# Autodesk Inventor assembly: сборка основание
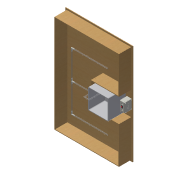
[picture p0: Inventor's stored thumbnail of the model, 180x180]
Saved by Autodesk Inventor 2021 (Build 250183000, 183)
## iProperties
Created: 2023-02-14
Part Number: сборка основание
Document SubType Name: Assembly
Designer: Tasya
Author: Tasya
## Documents named in this file (14)
- C:\Users\Tasya\Desktop\теплица\3D\Сборки iam\сборка основание.iam
- C:\Users\Tasya\Desktop\теплица\основание\основание.ipt
- C:\Users\Tasya\Desktop\теплица\основание\сосуд.ipt
- C:\Users\Tasya\Desktop\теплица\основание\стенка 1.ipt
- C:\Users\Tasya\Desktop\теплица\основание\стенка боковая.ipt
- C:\Users\Tasya\Desktop\теплица\основание\стенка 2.ipt
- C:\Users\Tasya\Desktop\теплица\основание\стенка 3.ipt
- C:\Users\Tasya\Desktop\теплица\основание\стенка 4.ipt
- C:\Users\Tasya\Desktop\теплица\емкость\шланг передний.ipt
- C:\Users\Tasya\Desktop\теплица\емкость\шланг боковой.ipt
- C:\Users\Tasya\Desktop\теплица\емкость\компановка емкость.iam
- C:\Users\Tasya\Desktop\теплица\емкость\змея.ipt
- C:\Users\Tasya\Desktop\теплица\емкость\соединитель 1.ipt
- C:\Users\Tasya\Desktop\теплица\емкость\соединитель 2.ipt
## Components (19 placed, 13 different names)
1. основание:1 — Угол:2, Угол:5, Заподлицо:1, Совмещение:50, Совмещение:51, Совмещение:54, Совмещение:55, Совмещение:56, Заподлицо:3, Совмещение:57, Совмещение:58, Совмещение:59, Совмещение:60, Совмещение:61, Совмещение:62, Совмещение:63, Совмещение:64, Совмещение:65, Совмещение:66, Совмещение:67, Совмещение:74, Угол:6, Угол:7, Угол:8, Совмещение:91, Совмещение:92, Совмещение:94, Совмещение:95, Совмещение:96, Совмещение:97, Совмещение:99, Совмещение:100
2. сосуд:1 — Заподлицо:1, Совмещение:50, Совмещение:51, Совмещение:75
3. шланг передний:1 — Совмещение:79, Совмещение:81, Совмещение:83, Совмещение:84
4. шланг передний:2 — Угол:2, Совмещение:78, Совмещение:82, Совмещение:87, Совмещение:89
5. шланг боковой:1 — Совмещение:85, Совмещение:86, Угол:8
6. шланг боковой:2 — Совмещение:88, Совмещение:90, Угол:7
7. компановка емкость:1 [sub-assembly] — Совмещение:91, Совмещение:92, Совмещение:93
8. змея:1 — Совмещение:47, Угол:5, Касательность:1, Совмещение:74, Совмещение:75, Совмещение:76, Совмещение:77, Совмещение:80
9. стенка 1:1 — Совмещение:54, Совмещение:55, Совмещение:56, Заподлицо:4
10. стенка 2:1 — Заподлицо:3, Совмещение:57, Совмещение:58
11. стенка боковая:1 — Совмещение:59, Совмещение:60, Совмещение:61
12. стенка 3:1 — Совмещение:62, Совмещение:63, Совмещение:64
13. стенка 4:1 — Совмещение:65, Совмещение:66, Совмещение:67, Касательность:1, Заподлицо:5
14. соединитель 1:1 — Совмещение:76, Угол:6, Совмещение:77, Совмещение:78, Совмещение:79, Совмещение:80, Совмещение:81, Совмещение:82
15. соединитель 2:1 — Совмещение:87, Совмещение:88, Совмещение:89, Совмещение:90
16. соединитель 2:2 — Совмещение:83, Совмещение:84, Совмещение:85, Совмещение:86
17. стенка 2:2 — Совмещение:96, Совмещение:97, Совмещение:98
18. стенка 3:2 — Совмещение:99, Заподлицо:5, Совмещение:100
19. стенка боковая:2 — Совмещение:94, Совмещение:95, Заподлицо:4, Совмещение:98
## Relationships (54: Mate 44, Angle 5, Flush 4, Tangent 1)
- Угол:2 [Angle] (0 deg): основание:1 ↔ шланг передний:2
- Совмещение:47 [Mate]: змея:1
- Угол:5 [Angle] (180 deg): основание:1 ↔ змея:1
- Заподлицо:1 [Flush]: основание:1 ↔ сосуд:1
- Совмещение:50 [Mate]: основание:1 ↔ сосуд:1
- Совмещение:51 [Mate]: основание:1 ↔ сосуд:1
- Совмещение:54 [Mate]: основание:1 ↔ стенка 1:1
- Совмещение:55 [Mate]: основание:1 ↔ стенка 1:1
- Совмещение:56 [Mate]: основание:1 ↔ стенка 1:1
- Заподлицо:3 [Flush]: основание:1 ↔ стенка 2:1
- Совмещение:57 [Mate]: основание:1 ↔ стенка 2:1
- Совмещение:58 [Mate]: основание:1 ↔ стенка 2:1
- Совмещение:59 [Mate]: основание:1 ↔ стенка боковая:1
- Совмещение:60 [Mate]: основание:1 ↔ стенка боковая:1
- Совмещение:61 [Mate]: основание:1 ↔ стенка боковая:1
- Совмещение:62 [Mate]: основание:1 ↔ стенка 3:1
- Совмещение:63 [Mate]: основание:1 ↔ стенка 3:1
- Совмещение:64 [Mate]: основание:1 ↔ стенка 3:1
- Совмещение:65 [Mate]: основание:1 ↔ стенка 4:1
- Совмещение:66 [Mate]: основание:1 ↔ стенка 4:1
- Совмещение:67 [Mate]: основание:1 ↔ стенка 4:1
- Касательность:1 [Tangent] (3 mm): змея:1 ↔ стенка 4:1
- Совмещение:74 [Mate] (71.5 mm): основание:1 ↔ змея:1
- Совмещение:75 [Mate] (7.5 mm): сосуд:1 ↔ змея:1
- Совмещение:76 [Mate]: змея:1 ↔ соединитель 1:1
- Угол:6 [Angle] (0 deg): основание:1 ↔ соединитель 1:1
- Совмещение:77 [Mate]: змея:1 ↔ соединитель 1:1
- Совмещение:78 [Mate]: шланг передний:2 ↔ соединитель 1:1
- Совмещение:79 [Mate]: шланг передний:1 ↔ соединитель 1:1
- Совмещение:80 [Mate] (-10 mm): змея:1 ↔ соединитель 1:1
- Совмещение:81 [Mate] (-10 mm): шланг передний:1 ↔ соединитель 1:1
- Совмещение:82 [Mate] (-10 mm): шланг передний:2 ↔ соединитель 1:1
- Совмещение:83 [Mate]: шланг передний:1 ↔ соединитель 2:2
- Совмещение:84 [Mate] (-10 mm): шланг передний:1 ↔ соединитель 2:2
- Совмещение:85 [Mate]: шланг боковой:1 ↔ соединитель 2:2
- Совмещение:86 [Mate] (-10 mm): шланг боковой:1 ↔ соединитель 2:2
- Совмещение:87 [Mate]: шланг передний:2 ↔ соединитель 2:1
- Совмещение:88 [Mate]: шланг боковой:2 ↔ соединитель 2:1
- Совмещение:89 [Mate] (-10 mm): шланг передний:2 ↔ соединитель 2:1
- Совмещение:90 [Mate] (-10 mm): шланг боковой:2 ↔ соединитель 2:1
- Угол:7 [Angle] (90 deg): основание:1 ↔ шланг боковой:2
- Угол:8 [Angle] (0 deg): основание:1 ↔ шланг боковой:1
- Совмещение:91 [Mate]: основание:1 ↔ компановка емкость:1
- Совмещение:92 [Mate]: основание:1 ↔ компановка емкость:1
- Совмещение:93 [Mate]: компановка емкость:1
- Совмещение:94 [Mate]: основание:1 ↔ стенка боковая:2
- Совмещение:95 [Mate]: основание:1 ↔ стенка боковая:2
- Заподлицо:4 [Flush]: стенка 1:1 ↔ стенка боковая:2
- Совмещение:96 [Mate]: основание:1 ↔ стенка 2:2
- Совмещение:97 [Mate]: основание:1 ↔ стенка 2:2
- Совмещение:98 [Mate]: стенка 2:2 ↔ стенка боковая:2
- Совмещение:99 [Mate]: основание:1 ↔ стенка 3:2
- Заподлицо:5 [Flush]: стенка 4:1 ↔ стенка 3:2
- Совмещение:100 [Mate]: основание:1 ↔ стенка 3:2
